# Autodesk Inventor assembly: CADAssembly2
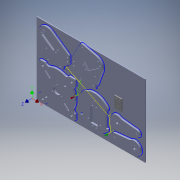
[picture p0: Inventor's stored thumbnail of the model, 180x180]
Saved by Autodesk Inventor 2016 (Build 200138000, 138)
## iProperties
Created: 2018-04-01
Part Number: CADAssembly2
Document SubType Name: Assembly
Designer: Nuwan
Sending System: SolidWorks 2014
Last Author: Nuwan
Last Saved: 2018-04-04
Author: Nuwan
## Documents named in this file (8)
- D:\Projects\Robot Arm\robort-arm\cad\CADAssembly2.iam
- D:\Projects\Robot Arm\robort-arm\cad\workpiece-base.ipt
- D:\Projects\Robot Arm\robort-arm\cad\base11.ipt
- D:\Projects\Robot Arm\robort-arm\cad\base12.ipt
- D:\Projects\Robot Arm\robort-arm\cad\link1.ipt
- D:\Projects\Robot Arm\robort-arm\cad\base01.ipt
- D:\Projects\Robot Arm\robort-arm\cad\inventor\base13.ipt
- D:\Projects\Robot Arm\robort-arm\cad\inventor\limit-holders.ipt
## Components (9 placed, 7 different names)
1. workpiece-base:2 — Mate:1, Mate:3, Mate:4
2. base11:1
3. base12:1
4. base12:2 — Mate:2
5. link1:1
6. link1:2
7. base01:1
8. base13:1 — Mate:1, Mate:2
9. limit-holders:2 — Mate:3, Mate:4
## Relationships (4: Mate 4)
- Mate:1: workpiece-base:2 ↔ base13:1
- Mate:2: base12:2 ↔ base13:1
- Mate:3: workpiece-base:2 ↔ limit-holders:2
- Mate:4: workpiece-base:2 ↔ limit-holders:2
